# Autodesk Inventor assembly: Assembly1
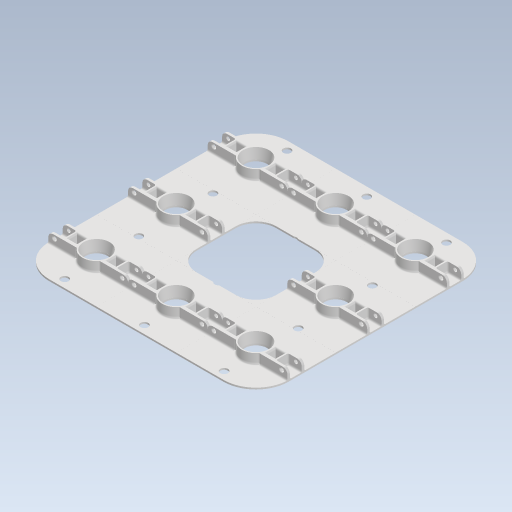
[picture p0: Inventor's stored thumbnail of the model, 512x512]
Saved by Autodesk Inventor 2023 (Build 270158000, 158)
## iProperties
Created: 2022-10-31
Part Number: Assembly1
Document SubType Name: Assembly
Designer: Dave
Author: Dave
## Documents named in this file (2)
- C:\Users\Dave\Documents\GrabCAD\Chalk Bot\Chalkbot1.0\Apparatus\V5\Assembly1.iam
- C:\Users\Dave\Documents\GrabCAD\Chalk Bot\Chalkbot1.0\Apparatus\V5\Base.ipt
## Components (9 placed, 1 different names)
1. Base:1
2. Base:2
3. Base:3
4. Base:4
5. Base:5
6. Base:6
7. Base:7
8. Base:8
9. Base:9
## Component patterns: (9 elements, first: Base:1)
